# Autodesk Inventor assembly: Electrical Board A
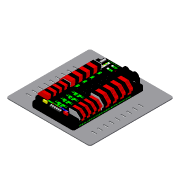
[picture p0: Inventor's stored thumbnail of the model, 180x180]
Saved by Autodesk Inventor 2015 (Build 190159000, 159)
## iProperties
Created: 2015-01-12
Part Number: Electrical Board A
Document SubType Name: Assembly
Designer: Peter
Author: Peter
## Documents named in this file (3)
- C:\Users\Noah\Desktop\FIRST-Team-1719-CAD-Team\2015 Robot CAD\Electrical\Electrical Board A.iam
- C:\Users\Noah\Desktop\FIRST-Team-1719-CAD-Team\2015 Robot CAD\Electrical\Power Board - Plate A.ipt
- C:\Users\Noah\Desktop\FIRST-Team-1719-CAD-Team\2015 Robot CAD\Imported Components\Power Distribution Board Assembly.ipt
## Components (2 placed, 2 different names)
1. Power Board - Plate A:1 — Mate:1, Mate:2, Insert:1
2. Power Distribution Board Assembly:1 — Mate:1, Mate:2, Insert:1
## Relationships (3: Mate 2, Insert 1)
- Mate:1: Power Board - Plate A:1 ↔ Power Distribution Board Assembly:1
- Mate:2: Power Board - Plate A:1 ↔ Power Distribution Board Assembly:1
- Insert:1: Power Board - Plate A:1 ↔ Power Distribution Board Assembly:1
